# Autodesk Inventor assembly: MQ-Collapsed-View
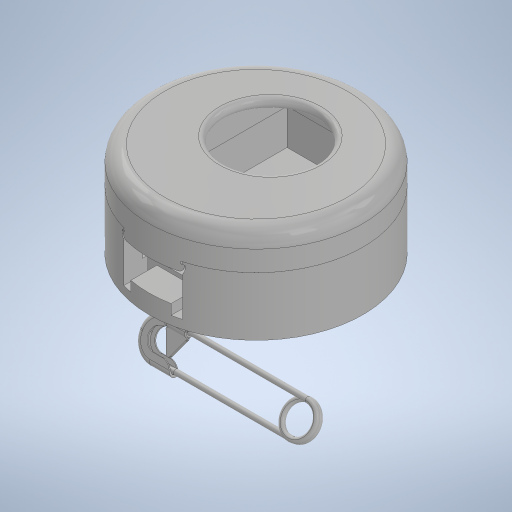
[picture p0: Inventor's stored thumbnail of the model, 512x512]
Saved by Autodesk Inventor 2023 (Build 270158000, 158)
## iProperties
Created: 2024-03-19
Part Number: MQ-Collapsed-View
Document SubType Name: Assembly
Designer: ongyu
Author: ongyu
## Documents named in this file (4)
- C:\Users\ongyu\OneDrive\Documents\Inventor\FYP\MQ-Shell\MQ-Collapsed-View.iam
- C:\Users\ongyu\OneDrive\Documents\Inventor\FYP\MQ-Shell\01 - MQ-Case-Btm.ipt
- C:\Users\ongyu\OneDrive\Documents\Inventor\FYP\MQ-Shell\02 - MQ-Case-Top.ipt
- C:\Users\ongyu\OneDrive\Documents\Inventor\FYP\MQ-Shell\05 - Safety-Pin.ipt
## Components (3 placed, 3 different names)
1. 01 - MQ-Case-Btm:1 — Flush:1, Mate:1, Flush:2, Insert:1, Mate:9
2. 02 - MQ-Case-Top:1 — Insert:1
3. 05 - Safety-Pin:1 — Mate:9, Flush:3
## Relationships (6: Flush 3, Mate 2, Insert 1)
- Flush:1: 01 - MQ-Case-Btm:1
- Mate:1: 01 - MQ-Case-Btm:1
- Flush:2: 01 - MQ-Case-Btm:1
- Insert:1: 01 - MQ-Case-Btm:1 ↔ 02 - MQ-Case-Top:1
- Mate:9 (15 mm): 01 - MQ-Case-Btm:1 ↔ 05 - Safety-Pin:1
- Flush:3: 05 - Safety-Pin:1
